# Autodesk Inventor assembly: wingpio-front-panel
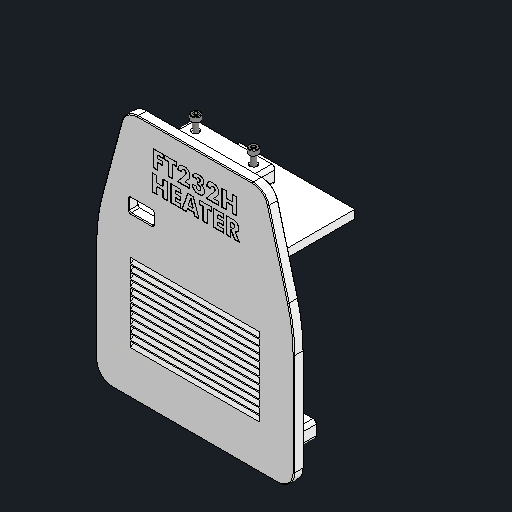
[picture p0: Inventor's stored thumbnail of the model, 512x512]
Saved by Autodesk Inventor 2026 (Build 300175050, 175E)
## iProperties
Created: 2026-03-04
Part Number: wingpio-front-panel
Document SubType Name: Assembly
Designer: kuzmin
Author: kuzmin
## Documents named in this file (7)
- C:\Users\queez\Dropbox\Drawings\PIHTI\ElectronicsBox\Win-GPIO-Box\wingpio-front-panel.iam
- C:\Users\queez\Dropbox\Drawings\PIHTI\ElectronicsBox\Win-GPIO-Box\front-panel.ipt
- C:\Users\queez\Dropbox\Drawings\PIHTI\ContentCenter\Fastners\M3-nut.ipt
- C:\Users\queez\Dropbox\Drawings\PIHTI\ContentCenter\Fastners\brass-insert-m3x5.ipt
- C:\Users\queez\Dropbox\Drawings\PIHTI\ContentCenter\Fastners\M3x10-SHCS.ipt
- C:\Users\queez\Dropbox\Drawings\PIHTI\ElectronicsBox\Win-GPIO-Box\modules-panel.ipt
- C:\Users\queez\Dropbox\Drawings\PIHTI\ElectronicsBox\Win-GPIO-Box\panel-mount.ipt
## Components (15 placed, 6 different names)
1. front-panel:1 — Rigid:1, Rigid:2, Rigid:3, Rigid:4, Rigid:5, Rigid:6, Rigid:7, Rigid:8, Rigid:9, Rigid:10, Mate:1, Flush:1, Rotational:1
2. brass-insert-m3x5:1 — Rigid:5
3. brass-insert-m3x5:2 — Rigid:6
4. modules-panel:1 — Mate:1, Flush:1
5. panel-mount:1 — Rotational:1, Rigid:11, Rigid:12
6. JIS B 1176 - Metric M3 x 10:5 — Rigid:12
7. JIS B 1176 - Metric M3 x 10:6 — Rigid:11
8. JIS B 1181 Style 1 - Metric A M3:1 — Rigid:1
9. JIS B 1181 Style 1 - Metric A M3:2 — Rigid:4
10. JIS B 1181 Style 1 - Metric A M3:3 — Rigid:3
11. JIS B 1181 Style 1 - Metric A M3:4 — Rigid:2
12. JIS B 1176 - Metric M3 x 10:1 — Rigid:7
13. JIS B 1176 - Metric M3 x 10:2 — Rigid:8
14. JIS B 1176 - Metric M3 x 10:3 — Rigid:9
15. JIS B 1176 - Metric M3 x 10:4 — Rigid:10
## Relationships (15: WeldJoint 12, Mate 1, Flush 1, RevoluteJoint 1)
- Rigid:1 [WeldJoint]: front-panel:1 ↔ JIS B 1181 Style 1 - Metric A M3:1
- Rigid:2 [WeldJoint]: front-panel:1 ↔ JIS B 1181 Style 1 - Metric A M3:4
- Rigid:3 [WeldJoint]: front-panel:1 ↔ JIS B 1181 Style 1 - Metric A M3:3
- Rigid:4 [WeldJoint]: front-panel:1 ↔ JIS B 1181 Style 1 - Metric A M3:2
- Rigid:5 [WeldJoint]: front-panel:1 ↔ brass-insert-m3x5:1
- Rigid:6 [WeldJoint]: front-panel:1 ↔ brass-insert-m3x5:2
- Rigid:7 [WeldJoint] (6 mm): front-panel:1 ↔ JIS B 1176 - Metric M3 x 10:1
- Rigid:8 [WeldJoint] (6 mm): front-panel:1 ↔ JIS B 1176 - Metric M3 x 10:2
- Rigid:9 [WeldJoint] (6 mm): front-panel:1 ↔ JIS B 1176 - Metric M3 x 10:3
- Rigid:10 [WeldJoint] (6 mm): front-panel:1 ↔ JIS B 1176 - Metric M3 x 10:4
- Mate:1: front-panel:1 ↔ modules-panel:1
- Flush:1 (4 mm): front-panel:1 ↔ modules-panel:1
- Rotational:1 [RevoluteJoint]: front-panel:1 ↔ panel-mount:1
- Rigid:11 [WeldJoint]: panel-mount:1 ↔ JIS B 1176 - Metric M3 x 10:6
- Rigid:12 [WeldJoint]: panel-mount:1 ↔ JIS B 1176 - Metric M3 x 10:5
